# Autodesk Inventor assembly: hang arm_MIR
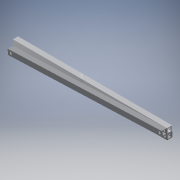
[picture p0: Inventor's stored thumbnail of the model, 180x180]
Saved by Autodesk Inventor 2016 (Build 200138000, 138)
## iProperties
Created: 2016-03-29
Part Number: hang arm_MIR
Document SubType Name: Assembly
Designer: gus
Author: gus
## Documents named in this file (4)
- \\Mac\Home\Desktop\1510-stronghold-CAD-master\hang arm 2.0\hang arm_MIR.iam
- \\Mac\Home\Desktop\1510-stronghold-CAD-master\hang arm 2.0\support bar_MIR.ipt
- \\Mac\Home\Desktop\1510-stronghold-CAD-master\hang arm 2.0\lower arm_MIR.ipt
- \\Mac\Home\Desktop\1510-stronghold-CAD-master\hang arm 2.0\upper arm_MIR.ipt
## Components (3 placed, 3 different names)
1. support bar_MIR:1 — Flush:1, Cylindrical:1
2. lower arm_MIR:1 — Flush:1, Mate:1, Cylindrical:1, Cylindrical:2
3. upper arm_MIR:1 — Mate:1, Cylindrical:2
## Relationships (4: Mate 2, CylindricalJoint 2)
- Flush:1 [Mate]: support bar_MIR:1 ↔ lower arm_MIR:1
- Mate:1: lower arm_MIR:1 ↔ upper arm_MIR:1
- Cylindrical:1: support bar_MIR:1 ↔ lower arm_MIR:1
- Cylindrical:2: lower arm_MIR:1 ↔ upper arm_MIR:1
